# Autodesk Inventor assembly: Bar Cabinet Assembly
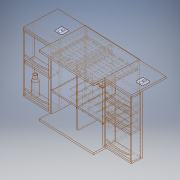
[picture p0: Inventor's stored thumbnail of the model, 180x180]
Saved by Autodesk Inventor 2016 (Build 200138000, 138)
## iProperties
Created: 2017-10-30
Part Number: Bar Cabinet Assembly
Document SubType Name: Assembly
Designer: mathaetaes
Author: mathaetaes
## Documents named in this file (14)
- E:\Projects\3D Printer\printer projects\My Designs\Bar Cabinet\Bar Cabinet Assembly.iam
- E:\Projects\3D Printer\printer projects\My Designs\Bar Cabinet\Left Side.ipt
- E:\Projects\3D Printer\printer projects\My Designs\Bar Cabinet\Top.ipt
- E:\Projects\3D Printer\printer projects\My Designs\Bar Cabinet\Horizontal Shelf.ipt
- E:\Projects\3D Printer\printer projects\My Designs\Bar Cabinet\Vertical Shelf.ipt
- E:\Projects\3D Printer\printer projects\My Designs\Bar Cabinet\Bottom.ipt
- E:\Projects\3D Printer\printer projects\My Designs\Bar Cabinet\Right Side.ipt
- E:\Projects\3D Printer\printer projects\My Designs\Bar Cabinet\Wine Glass Rack Full Assembly.iam
- E:\Projects\3D Printer\printer projects\My Designs\Bar Cabinet\Wine Rack Assembly.iam
- E:\Projects\3D Printer\printer projects\My Designs\Bar Cabinet\Drawer.iam
- E:\Projects\3D Printer\printer projects\My Designs\Bar Cabinet\Door.iam
- E:\Projects\3D Printer\printer projects\My Designs\Bar Cabinet\Door 2.iam
- E:\Projects\3D Printer\printer projects\My Designs\Bar Cabinet\Extension Shelves.ipt
- E:\Projects\3D Printer\printer projects\My Designs\Bar Cabinet\Back Panel.ipt
## Components (17 placed, 13 different names)
1. Left Side:1 — Flush:5, Mate:3, Flush:6, Mate:7, Flush:7, Mate:10, Mate:11, Mate:29, Flush:25, Mate:44, Mate:46, Mate:50, Rotational:2
2. Top:1 — Flush:5, Mate:6, Mate:9, Flush:11, Mate:10, Flush:30, Flush:32, Mate:51, Flush:36, Flush:38, Mate:54
3. Horizontal Shelf:1 — Mate:3, Mate:5, Flush:8, Mate:11, Flush:13
4. Vertical Shelf:1 — Mate:5, Mate:6, Flush:8, Mate:28, Mate:32, Flush:22, Mate:39, Mate:41, Mate:43
5. Bottom:1 — Flush:6, Mate:7, Flush:7, Mate:30, Mate:48, Mate:49, Flush:34
6. Right Side:1 — Mate:9, Flush:11, Flush:13, Mate:31, Flush:35, Mate:52, Rotational:1, Rotational:3
7. Wine Glass Rack Full Assembly:1 [sub-assembly] — Mate:42, Mate:43, Flush:27
8. Wine Glass Rack Full Assembly:2 [sub-assembly] — Mate:40, Mate:41, Flush:26
9. Wine Rack Assembly:1 [sub-assembly] — Mate:28, Mate:29, Mate:30
10. Wine Rack Assembly:2 [sub-assembly] — Mate:31, Mate:32, Flush:22
11. Drawer:1 [sub-assembly] — Mate:46
12. Horizontal Shelf:2 — Flush:25, Mate:39, Mate:40, Mate:42, Flush:26, Mate:44, Flush:27
13. Door 2:1 [sub-assembly] — Mate:48, Rotational:1
14. Door:1 [sub-assembly] — Mate:49, Rotational:2
15. Extension Shelves:1 — Flush:30, Flush:38, Mate:54
16. Extension Shelves:2 — Flush:32, Flush:36, Rotational:3
17. Back Panel:1 — Mate:50, Flush:34, Flush:35, Mate:51, Mate:52
## Relationships (44: Mate 25, Flush 16, RevoluteJoint 3)
- Flush:5: Left Side:1 ↔ Top:1
- Mate:3: Left Side:1 ↔ Horizontal Shelf:1
- Mate:5: Horizontal Shelf:1 ↔ Vertical Shelf:1
- Mate:6: Top:1 ↔ Vertical Shelf:1
- Flush:6: Left Side:1 ↔ Bottom:1
- Mate:7: Left Side:1 ↔ Bottom:1
- Flush:7: Left Side:1 ↔ Bottom:1
- Flush:8: Horizontal Shelf:1 ↔ Vertical Shelf:1
- Mate:9: Top:1 ↔ Right Side:1
- Flush:11: Top:1 ↔ Right Side:1
- Mate:10: Left Side:1 ↔ Top:1
- Mate:11: Left Side:1 ↔ Horizontal Shelf:1
- Flush:13: Horizontal Shelf:1 ↔ Right Side:1
- Mate:28: Vertical Shelf:1 ↔ Wine Rack Assembly:1
- Mate:29: Left Side:1 ↔ Wine Rack Assembly:1
- Mate:30: Bottom:1 ↔ Wine Rack Assembly:1
- Mate:31: Right Side:1 ↔ Wine Rack Assembly:2
- Mate:32: Vertical Shelf:1 ↔ Wine Rack Assembly:2
- Flush:22: Vertical Shelf:1 ↔ Wine Rack Assembly:2
- Flush:25: Left Side:1 ↔ Horizontal Shelf:2
- Mate:39: Vertical Shelf:1 ↔ Horizontal Shelf:2
- Mate:40: Wine Glass Rack Full Assembly:2 ↔ Horizontal Shelf:2
- Mate:41 (3.175 mm): Vertical Shelf:1 ↔ Wine Glass Rack Full Assembly:2
- Mate:42: Wine Glass Rack Full Assembly:1 ↔ Horizontal Shelf:2
- Mate:43 (3.175 mm): Vertical Shelf:1 ↔ Wine Glass Rack Full Assembly:1
- Flush:26: Wine Glass Rack Full Assembly:2 ↔ Horizontal Shelf:2
- Mate:44: Left Side:1 ↔ Horizontal Shelf:2
- Flush:27: Wine Glass Rack Full Assembly:1 ↔ Horizontal Shelf:2
- Mate:46 (6.35 mm): Left Side:1 ↔ Drawer:1
- Mate:48: Bottom:1 ↔ Door 2:1
- Mate:49: Bottom:1 ↔ Door:1
- Flush:30: Top:1 ↔ Extension Shelves:1
- Flush:32: Top:1 ↔ Extension Shelves:2
- Mate:50: Left Side:1 ↔ Back Panel:1
- Flush:34: Bottom:1 ↔ Back Panel:1
- Flush:35: Right Side:1 ↔ Back Panel:1
- Mate:51: Top:1 ↔ Back Panel:1
- Mate:52: Right Side:1 ↔ Back Panel:1
- Rotational:1 [RevoluteJoint]: Right Side:1 ↔ Door 2:1
- Rotational:2 [RevoluteJoint]: Left Side:1 ↔ Door:1
- Flush:36: Top:1 ↔ Extension Shelves:2
- Rotational:3 [RevoluteJoint]: Right Side:1 ↔ Extension Shelves:2
- Flush:38: Top:1 ↔ Extension Shelves:1
- Mate:54: Top:1 ↔ Extension Shelves:1
